# Autodesk Inventor assembly: Chassis and wheels assembly
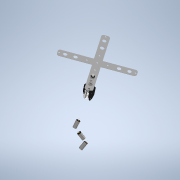
[picture p0: Inventor's stored thumbnail of the model, 180x180]
Saved by Autodesk Inventor 2020 (Build 240168000, 168)
## iProperties
Created: 2022-07-01
Part Number: Chassis and wheels assembly
Document SubType Name: Assembly
Designer: karimi2
Author: karimi2
## Documents named in this file (5)
- C:\Users\karimi2\Documents\PROJECT\src\Chassis and wheels assembly.iam
- C:\Users\karimi2\Documents\PROJECT\src\chassisPart1.ipt
- C:\Users\karimi2\Documents\PROJECT\src\GearedDCmotor.ipt
- C:\Users\karimi2\Documents\PROJECT\src\Wheel Assembly.iam
- C:\Users\karimi2\Documents\PROJECT\src\Chassis and wheels assembly\Design Accelerator\Synchronous Belts Transmission2.iam
## Components (8 placed, 4 different names)
1. chassisPart1:1 — Rigid:1, Rigid:2, Rigid:3, Rigid:4
2. chassisPart1:2 — Rigid:1
3. GearedDCmotor:1 — Rigid:2, Mate:1
4. GearedDCmotor:2
5. GearedDCmotor:3
6. GearedDCmotor:4
7. Wheel Assembly:1 [sub-assembly] — Rigid:3, Rigid:4, Rotational:1
8. Synchronous Belts Transmission:1 [sub-assembly] — Rotational:1, Mate:1
## Relationships (6: WeldJoint 4, RevoluteJoint 1, Mate 1)
- Rigid:1 [WeldJoint]: chassisPart1:1 ↔ chassisPart1:2
- Rigid:2 [WeldJoint]: chassisPart1:1 ↔ GearedDCmotor:1
- Rigid:3 [WeldJoint] (4.5 mm): chassisPart1:1 ↔ Wheel Assembly:1
- Rigid:4 [WeldJoint] (3.5 mm): chassisPart1:1 ↔ Wheel Assembly:1
- Rotational:1 [RevoluteJoint] (10 mm): Wheel Assembly:1 ↔ Synchronous Belts Transmission:1
- Mate:1: GearedDCmotor:1 ↔ Synchronous Belts Transmission:1
